# Autodesk Inventor assembly: mainflap
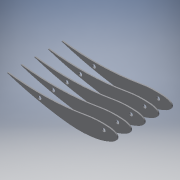
[picture p0: Inventor's stored thumbnail of the model, 180x180]
Saved by Autodesk Inventor 2018.2 (Build 222227000, 227)
## iProperties
Created: 2018-03-14
Part Number: mainflap
Material: 一般
Document SubType Name: Assembly
Designer: ku_sk
Author: ku_sk
## Documents named in this file (2)
- C:\Users\ku_sk\Documents\Inventor\Aero\KS-15\Rr.wing\parts\mainflap\mainflap.iam
- C:\Users\ku_sk\Documents\Inventor\Aero\KS-15\Rr.wing\parts\flap_m.ipt
## Components (5 placed, 1 different names)
1. flap_m:1 — メイト:3, メイト:7, メイト:9
2. flap_m:2 — メイト:2, メイト:3, メイト:6, メイト:7, メイト:8, メイト:9
3. flap_m:3 — フラッシュ:1, メイト:1, メイト:2, メイト:4, メイト:6, メイト:8, メイト:10, メイト:11
4. flap_m:4 — メイト:4, メイト:5, メイト:10, メイト:11, メイト:12, メイト:13
5. flap_m:5 — メイト:5, メイト:12, メイト:13
## Relationships (14: Mate 13, Flush 1)
- フラッシュ:1 [Flush]: flap_m:3
- メイト:1 [Mate]: flap_m:3
- メイト:2 [Mate] (41.5 mm): flap_m:2 ↔ flap_m:3
- メイト:3 [Mate] (41.5 mm): flap_m:1 ↔ flap_m:2
- メイト:4 [Mate] (41.5 mm): flap_m:3 ↔ flap_m:4
- メイト:5 [Mate] (41.5 mm): flap_m:4 ↔ flap_m:5
- メイト:6 [Mate]: flap_m:2 ↔ flap_m:3
- メイト:7 [Mate]: flap_m:1 ↔ flap_m:2
- メイト:8 [Mate]: flap_m:2 ↔ flap_m:3
- メイト:9 [Mate]: flap_m:1 ↔ flap_m:2
- メイト:10 [Mate]: flap_m:3 ↔ flap_m:4
- メイト:11 [Mate]: flap_m:3 ↔ flap_m:4
- メイト:12 [Mate]: flap_m:4 ↔ flap_m:5
- メイト:13 [Mate]: flap_m:4 ↔ flap_m:5
